# Autodesk Inventor assembly: cellSTORM_v5
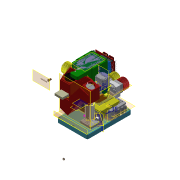
[picture p0: Inventor's stored thumbnail of the model, 180x180]
Saved by Autodesk Inventor 2022 (Build 260153000, 153)
## iProperties
Created: 2020-04-25
Part Number: cellSTORM_v5
Document SubType Name: Assembly
Designer: diederichbenedict
Author: diederichbenedict
## Documents named in this file (23)
- C:\Users\Muriel\Documents\GitHub\cellstorm\INVENTOR\cellSTORM_v6.iam
- C:\Users\Muriel\Documents\GitHub\cellstorm\INVENTOR\00_XY_stage-CHUO_SEIKI_LD-647-R1.iam
- C:\Users\Muriel\Documents\GitHub\cellstorm\INVENTOR\cellSTORM_laserbeam.ipt
- C:\Users\Muriel\Documents\GitHub\cellstorm\INVENTOR\02_Nanoscopy_Chip.ipt
- C:\Users\Muriel\Documents\GitHub\cellstorm\INVENTOR\00_Ballmagnets_5mm.ipt
- C:\Users\Muriel\Documents\GitHub\cellstorm\INVENTOR\00_Huawei_P20.ipt
- C:\Users\Muriel\Documents\GitHub\cellstorm\INVENTOR\cellSTORM_Base_v0_R1.ipt
- C:\Users\Muriel\Documents\GitHub\cellstorm\INVENTOR\00_KES400.iam
- C:\Users\Muriel\Documents\GitHub\cellstorm\INVENTOR\cellSTORM_v5_laserstage.ipt
- C:\Users\Muriel\Documents\GitHub\cellstorm\INVENTOR\cellSTORM_v5_cellphonestage.ipt
- C:\Users\Muriel\Documents\GitHub\cellstorm\INVENTOR\cellSTORM_v5_microsocpe.iam
- C:\Users\Muriel\Documents\GitHub\cellstorm\INVENTOR\cellSTORM_v5_microscope_cover.ipt
- C:\Users\Muriel\Documents\GitHub\cellstorm\INVENTOR\00_chip_01_old.ipt
- C:\Users\Muriel\Documents\GitHub\cellstorm\INVENTOR\cellSTORM_v5_chiptray_old_0.ipt
- C:\Users\Muriel\Documents\GitHub\cellstorm\INVENTOR\cellSTORM_v5_chiptry_clamp.ipt
- C:\Users\Muriel\Documents\GitHub\cellstorm\INVENTOR\00_Laser_532nm_200mw.ipt
- C:\Users\Muriel\Documents\GitHub\cellstorm\INVENTOR\00_LN680-Step.ipt
- C:\Users\Muriel\Documents\GitHub\cellstorm\INVENTOR\cellSTORM_v5_motorblock.ipt
- C:\Users\Muriel\Documents\GitHub\cellstorm\INVENTOR\cellSTORM_v5_cellphone_craddle.ipt
- C:\Users\Muriel\Documents\GitHub\cellstorm\INVENTOR\Assembly_Nema_Motor_attachement_for_XYstage.iam
- C:\Users\Muriel\Documents\GitHub\cellstorm\INVENTOR\00_RGB_Laser_converted.iam
- C:\Users\Muriel\Documents\GitHub\cellstorm\INVENTOR\00_Arduino_CNC_Assembly.iam
- C:\Users\diederichbenedict\Dropbox\cellSTORM\cellSTORM_v6.iam
## Components (25 placed, 21 different names)
1. 00_XY_stage-CHUO_SEIKI_LD-647-R1:1 [sub-assembly] — Insert:1, Angle:1, Insert:6, Angle:5, Flush:10, Flush:11
2. cellSTORM_laserbeam:1 — Insert:3, Insert:7, Insert:16, Passend:25
3. 02_Nanoscopy_Chip:1 — Insert:3, Angle:2
4. 00_Ballmagnets_5mm:1
5. 00_Ballmagnets_5mm:2
6. 00_Ballmagnets_5mm:3
7. cellSTORM_Base_v0_R1:1 — Insert:1, Angle:1, Angle:2, Flush:23
8. 00_XY_stage-CHUO_SEIKI_LD-647-R1:2 [sub-assembly] — Insert:6, Angle:5, Flush:12, Flush:13, Insert:17, Mate:26
9. 00_KES400:1 [sub-assembly] — Insert:7
10. cellSTORM_v5_laserstage:1 — Flush:10, Flush:11, Winkel:6, Fluchtend:26, Insert:18
11. cellSTORM_v5_cellphonestage:1 — Flush:12, Flush:13, Mate:10, Flush:14, Mate:24, Fluchtend:27, Flush:28, Flush:29
12. cellSTORM_v5_microsocpe:1 [sub-assembly] — Mate:10, Flush:14, Flush:15, Flush:16, Mate:23, Fluchtend:27
13. cellSTORM_v5_microscope_cover:1 — Flush:15, Flush:16
14. 00_Huawei_P20:1 — Mate:23, Mate:24, Flush:32
15. 00_chip_01_old:1 — Flush:22, Insert:16
16. cellSTORM_v5_chiptray_old_0:1 — Flush:22, Flush:23, Flush:24, Flush:25
17. cellSTORM_v5_chiptry_clamp:1 — Flush:24, Flush:25
18. 00_Laser_532nm_200mw:1 — Passend:25, Winkel:6, Fluchtend:26
19. 00_LN680-Step:1
20. cellSTORM_v5_motorblock:1 — Flush:28, Flush:29
21. cellSTORM_v5_cellphone_craddle:1 — Flush:32
22. Assembly_Nema_Motor_attachement_for_XYstage:1 [sub-assembly] — Insert:17
23. Assembly_Nema_Motor_attachement_for_XYstage:2 [sub-assembly] — Mate:26
24. 00_RGB_Laser_converted:1 [sub-assembly] — Insert:18
25. 00_Arduino_CNC_Assembly:1 [sub-assembly]
## Relationships (32: Flush 16, Insert 7, Mate 5, Angle 4)
- Insert:1: 00_XY_stage-CHUO_SEIKI_LD-647-R1:1 ↔ cellSTORM_Base_v0_R1:1
- Angle:1 (90 deg): 00_XY_stage-CHUO_SEIKI_LD-647-R1:1 ↔ cellSTORM_Base_v0_R1:1
- Insert:3 (5 mm): cellSTORM_laserbeam:1 ↔ 02_Nanoscopy_Chip:1
- Angle:2 (180 deg): 02_Nanoscopy_Chip:1 ↔ cellSTORM_Base_v0_R1:1
- Insert:6 (6 mm): 00_XY_stage-CHUO_SEIKI_LD-647-R1:1 ↔ 00_XY_stage-CHUO_SEIKI_LD-647-R1:2
- Angle:5 (180 deg): 00_XY_stage-CHUO_SEIKI_LD-647-R1:1 ↔ 00_XY_stage-CHUO_SEIKI_LD-647-R1:2
- Insert:7: cellSTORM_laserbeam:1 ↔ 00_KES400:1
- Flush:10: 00_XY_stage-CHUO_SEIKI_LD-647-R1:1 ↔ cellSTORM_v5_laserstage:1
- Flush:11: 00_XY_stage-CHUO_SEIKI_LD-647-R1:1 ↔ cellSTORM_v5_laserstage:1
- Flush:12: 00_XY_stage-CHUO_SEIKI_LD-647-R1:2 ↔ cellSTORM_v5_cellphonestage:1
- Flush:13: 00_XY_stage-CHUO_SEIKI_LD-647-R1:2 ↔ cellSTORM_v5_cellphonestage:1
- Mate:10: cellSTORM_v5_cellphonestage:1 ↔ cellSTORM_v5_microsocpe:1
- Flush:14: cellSTORM_v5_cellphonestage:1 ↔ cellSTORM_v5_microsocpe:1
- Flush:15: cellSTORM_v5_microsocpe:1 ↔ cellSTORM_v5_microscope_cover:1
- Flush:16: cellSTORM_v5_microsocpe:1 ↔ cellSTORM_v5_microscope_cover:1
- Mate:23: cellSTORM_v5_microsocpe:1 ↔ 00_Huawei_P20:1
- Mate:24: cellSTORM_v5_cellphonestage:1 ↔ 00_Huawei_P20:1
- Flush:22: 00_chip_01_old:1 ↔ cellSTORM_v5_chiptray_old_0:1
- Flush:23 (10 mm): cellSTORM_Base_v0_R1:1 ↔ cellSTORM_v5_chiptray_old_0:1
- Insert:16: cellSTORM_laserbeam:1 ↔ 00_chip_01_old:1
- Flush:24: cellSTORM_v5_chiptray_old_0:1 ↔ cellSTORM_v5_chiptry_clamp:1
- Flush:25: cellSTORM_v5_chiptray_old_0:1 ↔ cellSTORM_v5_chiptry_clamp:1
- Passend:25 [Mate]: cellSTORM_laserbeam:1 ↔ 00_Laser_532nm_200mw:1
- Winkel:6 [Angle] (180 deg): cellSTORM_v5_laserstage:1 ↔ 00_Laser_532nm_200mw:1
- Fluchtend:26 [Flush] (-15 mm): cellSTORM_v5_laserstage:1 ↔ 00_Laser_532nm_200mw:1
- Fluchtend:27 [Flush]: cellSTORM_v5_cellphonestage:1 ↔ cellSTORM_v5_microsocpe:1
- Flush:28: cellSTORM_v5_cellphonestage:1 ↔ cellSTORM_v5_motorblock:1
- Flush:29: cellSTORM_v5_cellphonestage:1 ↔ cellSTORM_v5_motorblock:1
- Flush:32: 00_Huawei_P20:1 ↔ cellSTORM_v5_cellphone_craddle:1
- Insert:17 (10 mm): 00_XY_stage-CHUO_SEIKI_LD-647-R1:2 ↔ Assembly_Nema_Motor_attachement_for_XYstage:1
- Mate:26 (5 mm): 00_XY_stage-CHUO_SEIKI_LD-647-R1:2 ↔ Assembly_Nema_Motor_attachement_for_XYstage:2
- Insert:18: cellSTORM_v5_laserstage:1 ↔ 00_RGB_Laser_converted:1
